# Autodesk Inventor assembly: JF-AT-TM0006
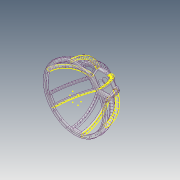
[picture p0: Inventor's stored thumbnail of the model, 180x180]
Saved by Autodesk Inventor 2015 SP1 (Build 190203100, 203)
## iProperties
Created: 2010-10-27
Part Number: JF-AT-TM0006
Document SubType Name: Assembly
Designer: D Flickinger
Vendor: HHMI: JRC - ID&F
Description: BOWL FRAME FOR MOUSE TREADMILL
ALTERED ITEM DESCRIPTION: N/A
DESIGN DEPARTMENT: HHMI: JRC - ID&F
Revision Number: 0
## Documents named in this file (4)
- C:\_WORKSPACE\DATA\COLLABORATION\SVOBODA LAB\MOUSE POSITIONING SYSTEMS\MCAD\BALL SETUP\16 inch ball treadmill assembly.iam
- C:\_WORKSPACE\DATA\COLLABORATION\SVOBODA LAB\MOUSE POSITIONING SYSTEMS\MCAD\BALL SETUP\Ball_Rig\16 inch ball treadmill frame base v2.ipt
- C:\_WORKSPACE\DATA\COLLABORATION\SVOBODA LAB\MOUSE POSITIONING SYSTEMS\MCAD\BALL SETUP\Ball_Rig\16 inch ball treadmill frame v2.ipt
- C:\_WORKSPACE\DATA\COLLABORATION\SVOBODA LAB\MOUSE POSITIONING SYSTEMS\MCAD\BALL SETUP\Ball_Rig\16 inch ball treadmill top ring v2.ipt
## Components (8 placed, 3 different names)
1. 16 inch ball treadmill frame base v2:1 — Mate:1, Mate:2, Mate:3, Mate:4, Mate:5, Mate:6, Mate:7, Mate:8, Mate:9, Mate:10, Mate:11, Mate:12, Mate:13, Mate:14, Mate:15, Mate:16, Mate:17, Mate:18
2. 16 inch ball treadmill frame v2:1 — Mate:10, Mate:11, Mate:12, Mate:19, Tangent:1
3. 16 inch ball treadmill frame v2:2 — Mate:4, Mate:5, Mate:6
4. 16 inch ball treadmill frame v2:3 — Mate:1, Mate:2, Mate:3
5. 16 inch ball treadmill frame v2:4 — Mate:7, Mate:8, Mate:9
6. 16 inch ball treadmill frame v2:5 — Mate:13, Mate:14, Mate:15, Tangent:2
7. 16 inch ball treadmill frame v2:6 — Mate:16, Mate:17, Mate:18
8. 16 inch ball treadmill top ring v2:1 — Mate:19, Tangent:1, Tangent:2
## Relationships (21: Mate 19, Tangent 2)
- Mate:1: 16 inch ball treadmill frame base v2:1 ↔ 16 inch ball treadmill frame v2:3
- Mate:2: 16 inch ball treadmill frame base v2:1 ↔ 16 inch ball treadmill frame v2:3
- Mate:3: 16 inch ball treadmill frame base v2:1 ↔ 16 inch ball treadmill frame v2:3
- Mate:4: 16 inch ball treadmill frame base v2:1 ↔ 16 inch ball treadmill frame v2:2
- Mate:5: 16 inch ball treadmill frame base v2:1 ↔ 16 inch ball treadmill frame v2:2
- Mate:6: 16 inch ball treadmill frame base v2:1 ↔ 16 inch ball treadmill frame v2:2
- Mate:7: 16 inch ball treadmill frame base v2:1 ↔ 16 inch ball treadmill frame v2:4
- Mate:8: 16 inch ball treadmill frame base v2:1 ↔ 16 inch ball treadmill frame v2:4
- Mate:9: 16 inch ball treadmill frame base v2:1 ↔ 16 inch ball treadmill frame v2:4
- Mate:10: 16 inch ball treadmill frame base v2:1 ↔ 16 inch ball treadmill frame v2:1
- Mate:11: 16 inch ball treadmill frame base v2:1 ↔ 16 inch ball treadmill frame v2:1
- Mate:12: 16 inch ball treadmill frame base v2:1 ↔ 16 inch ball treadmill frame v2:1
- Mate:13: 16 inch ball treadmill frame base v2:1 ↔ 16 inch ball treadmill frame v2:5
- Mate:14: 16 inch ball treadmill frame base v2:1 ↔ 16 inch ball treadmill frame v2:5
- Mate:15: 16 inch ball treadmill frame base v2:1 ↔ 16 inch ball treadmill frame v2:5
- Mate:16: 16 inch ball treadmill frame base v2:1 ↔ 16 inch ball treadmill frame v2:6
- Mate:17: 16 inch ball treadmill frame base v2:1 ↔ 16 inch ball treadmill frame v2:6
- Mate:18: 16 inch ball treadmill frame base v2:1 ↔ 16 inch ball treadmill frame v2:6
- Mate:19: 16 inch ball treadmill frame v2:1 ↔ 16 inch ball treadmill top ring v2:1
- Tangent:1: 16 inch ball treadmill frame v2:1 ↔ 16 inch ball treadmill top ring v2:1
- Tangent:2: 16 inch ball treadmill frame v2:5 ↔ 16 inch ball treadmill top ring v2:1
